# Autodesk Inventor assembly: lcdAssembly
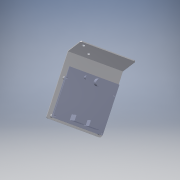
[picture p0: Inventor's stored thumbnail of the model, 180x180]
Saved by Autodesk Inventor 2017 (Build 210142000, 142)
## iProperties
Created: 2018-07-05
Part Number: lcdAssembly
Document SubType Name: Assembly
Designer: UnKnoWn
Author: UnKnoWn
## Documents named in this file (4)
- I:\3d Printer stuff\Ender 3\Ender3 working files\Ender-3 Mechanical\STP\lcdAssembly.iam
- I:\3d Printer stuff\Ender 3\Ender3 working files\Ender-3 Mechanical\STP\LCD support.ipt
- I:\3d Printer stuff\Ender 3\Ender3 working files\Ender-3 Mechanical\STP\lcd.ipt
- I:\3d Printer stuff\Ender 3\Ender3 working files\Ender-3 Mechanical\STP\lcd Knob.ipt
## Components (3 placed, 3 different names)
1. LCD support:1
2. lcd:1 — Mate:1, Mate:2
3. lcd Knob:1 — Mate:1, Mate:2
## Relationships (2: Mate 2)
- Mate:1: lcd:1 ↔ lcd Knob:1
- Mate:2: lcd:1 ↔ lcd Knob:1
